# Autodesk Inventor assembly: feed
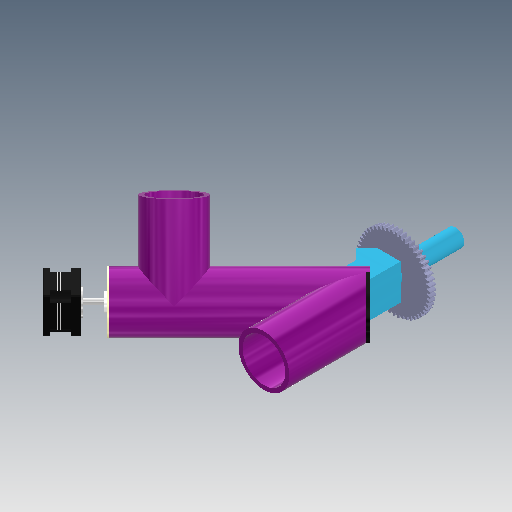
[picture p0: Inventor's stored thumbnail of the model, 512x512]
Saved by Autodesk Inventor 2020 (Build 240168000, 168)
## iProperties
Created: 2020-06-18
Part Number: feed
Document SubType Name: Assembly
Designer: pc-konvi
Author: pc-konvi
## Documents named in this file (7)
- C:\Users\pc-konvi\Documents\Lobola\open_source_scrabble\lobola - rapid prototype\feed.iam
- C:\Users\pc-konvi\Documents\Lobola\open_source_scrabble\lobola - rapid prototype\Feed_pin.ipt
- C:\Users\pc-konvi\Documents\Lobola\open_source_scrabble\lobola - rapid prototype\feed_cover.ipt
- C:\Users\pc-konvi\Documents\Lobola\open_source_scrabble\lobola - rapid prototype\feed_gear_assembly\Design Accelerator\Spur Gear21.ipt
- C:\Users\pc-konvi\Documents\Lobola\open_source_scrabble\lobola - rapid prototype\arc_screw.ipt
- C:\Users\pc-konvi\Documents\Lobola\open_source_scrabble\lobola - rapid prototype\NEMA14.ipt
- C:\Users\pc-konvi\Documents\Lobola\open_source_scrabble\lobola - rapid prototype\feed_lid.ipt
## Components (6 placed, 6 different names)
1. Feed_pin:1 — Mate:1, Mate:2, Mate:3, Mate:4, Mate:5, Mate:6, Mate:10
2. feed_cover:1 — Mate:3, Mate:4, Mate:7, Mate:8, Mate:9, Mate:11, Flush:1, Mate:12, Mate:14
3. Spur Gear2:1 — Mate:5, Mate:6
4. arc_screw:1 — Mate:7, Mate:8, Mate:13
5. NEMA14:1 — Mate:9, Mate:11, Mate:12
6. feed_lid:1 — Mate:13, Mate:14
## Relationships (15: Mate 14, Flush 1)
- Mate:1: Feed_pin:1
- Mate:2: Feed_pin:1
- Mate:3: Feed_pin:1 ↔ feed_cover:1
- Mate:4: Feed_pin:1 ↔ feed_cover:1
- Mate:5: Feed_pin:1 ↔ Spur Gear2:1
- Mate:6 (4 mm): Feed_pin:1 ↔ Spur Gear2:1
- Mate:7: feed_cover:1 ↔ arc_screw:1
- Mate:8: feed_cover:1 ↔ arc_screw:1
- Mate:9: feed_cover:1 ↔ NEMA14:1
- Mate:10: Feed_pin:1
- Mate:11: feed_cover:1 ↔ NEMA14:1
- Flush:1: feed_cover:1
- Mate:12 (20 mm): feed_cover:1 ↔ NEMA14:1
- Mate:13: arc_screw:1 ↔ feed_lid:1
- Mate:14: feed_cover:1 ↔ feed_lid:1
